# Autodesk Inventor assembly: The Nosecone Mould
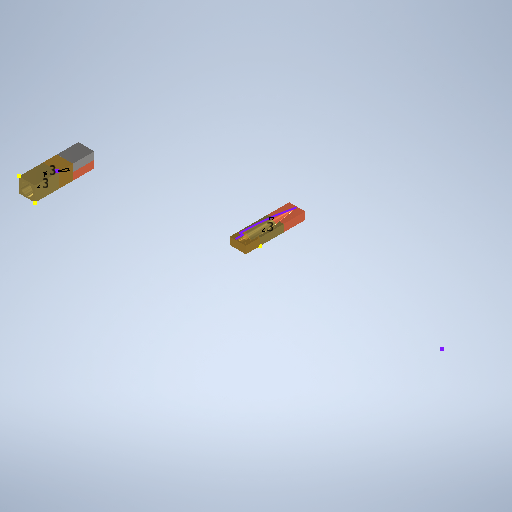
[picture p0: Inventor's stored thumbnail of the model, 512x512]
Saved by Autodesk Inventor 2025 (Build 290162000, 162)
## iProperties
Created: 2024-06-06
Part Number: The Nosecone Mould
Document SubType Name: Assembly
Designer: agnes
Author: agnes
## Documents named in this file (7)
- C:\Users\agnes\OneDrive\Documents\Nakuja\Nosecone mould\The Nosecone Mould.iam
- C:\Users\agnes\OneDrive\Documents\Nakuja\Nosecone mould\First negative.ipt
- C:\Users\agnes\OneDrive\Documents\Nakuja\Nosecone mould\First.ipt
- C:\Users\agnes\OneDrive\Documents\Nakuja\Nosecone mould\Second negative.ipt
- C:\Users\agnes\OneDrive\Documents\Nakuja\Nosecone mould\Second.ipt
- C:\Users\agnes\OneDrive\Documents\Nakuja\Nosecone mould\Third negative.ipt
- C:\Users\agnes\OneDrive\Documents\Nakuja\Nosecone mould\Third.ipt
## Components (9 placed, 6 different names)
1. First negative:1 — Mate:3, Mate:4, Mate:7, Mate:8
2. First:1 — Mate:5, Mate:6, Mate:10
3. Second negative:1 — Mate:1, Mate:2, Mate:5
4. Second:1 — Mate:1, Mate:2, Mate:3, Mate:4, Mate:6
5. Third:1 — Mate:9, Mate:10
6. Third negative:1 — Mate:7, Mate:8, Mate:9
7. First negative:2 — Mate:13, Mate:14
8. Second negative:2 — Mate:11, Mate:12, Mate:13, Mate:14
9. Third negative:2 — Mate:11, Mate:12
## Relationships (14: Mate 14)
- Mate:1: Second negative:1 ↔ Second:1
- Mate:2: Second negative:1 ↔ Second:1
- Mate:3: First negative:1 ↔ Second:1
- Mate:4: First negative:1 ↔ Second:1
- Mate:5: First:1 ↔ Second negative:1
- Mate:6: First:1 ↔ Second:1
- Mate:7: First negative:1 ↔ Third negative:1
- Mate:8: First negative:1 ↔ Third negative:1
- Mate:9: Third:1 ↔ Third negative:1
- Mate:10: First:1 ↔ Third:1
- Mate:11: Second negative:2 ↔ Third negative:2
- Mate:12: Second negative:2 ↔ Third negative:2
- Mate:13: First negative:2 ↔ Second negative:2
- Mate:14: First negative:2 ↔ Second negative:2
